# Autodesk Inventor assembly: GP9-100
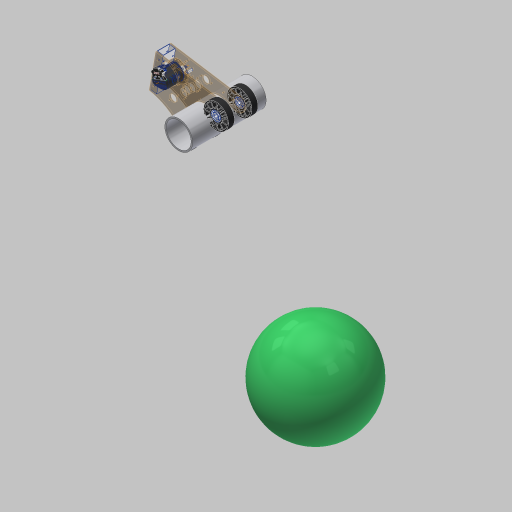
[picture p0: Inventor's stored thumbnail of the model, 512x512]
Saved by Autodesk Inventor 2023.5 (Build 275446000, 446)
## iProperties
Created: 2025-02-27
Part Number: GP9-100
Document SubType Name: Assembly
Designer: dlangdon
Author: dlangdon
## Documents named in this file (11)
- C:\Users\slick\OneDrive\Desktop\2025-ReefScape---CAD\Gripper\GP9\GP9-100.iam
- C:\Users\slick\OneDrive\Desktop\2025-ReefScape---CAD\Gripper\GP9\GP9-001.ipt
- C:\Users\slick\OneDrive\Desktop\2025-ReefScape---CAD\Gripper\GP9\GP9-002.ipt
- C:\Users\slick\OneDrive\Desktop\2025-ReefScape---CAD\Gripper\GP9\GP9-004.ipt
- C:\Users\slick\OneDrive\Desktop\2025-ReefScape---CAD\Gripper\GP9\GP9-003.ipt
- C:\Users\slick\OneDrive\Desktop\2025-ReefScape---CAD\Gripper\GP6\GP6-006.ipt
- C:\Users\slick\OneDrive\Desktop\2025-ReefScape---CAD\COMMON PARTS\MOTORS\Kracken with Cover and Boards.iam
- C:\Users\slick\OneDrive\Desktop\2025-ReefScape---CAD\COMMON PARTS\PULLEYS\gt2\16T Falcon GT216T x 9mm Wide Double Flange Aluminum Pulley (GT2 3mm, Falcon Motor)  (217-6924).iam
- C:\Users\slick\OneDrive\Desktop\2025-ReefScape---CAD\COMMON PARTS\WHEELS\am-3480 4IN 500Hex Bore Compliant Wheel REV2 (1).iam
- C:\Users\slick\OneDrive\Desktop\2025-ReefScape---CAD\Field Items\Game Pieces\GE-25500.ipt
- C:\Users\slick\OneDrive\Desktop\2025-ReefScape---CAD\Field Items\Game Pieces\GE-25501.ipt
## Components (14 placed, 10 different names)
1. GP9-001:1 — Insert:1, Insert:2, Insert:7, Insert:8, Mate:1, Mate:4
2. GP9-002:1 — Insert:3, Insert:4, Mate:2, Mate:3, Mate:5
3. GP9-004:1 — Insert:1, Insert:2, Insert:3, Insert:4
4. GP9-003:1 — Insert:5, Insert:6, Insert:10, Insert:11
5. GP6-006:1 — Insert:6, Insert:7
6. GP6-006:2 — Insert:5, Insert:8
7. Kracken with Cover and Boards:1 [sub-assembly] — Insert:9, Insert:10, Insert:11
8. 16T Falcon GT216T x 9mm Wide Double Flange Aluminum Pulley (GT2 3mm, Falcon Motor)  (217-6924):1 [sub-assembly] — Insert:9
9. am-3480 4IN 500Hex Bore Compliant Wheel REV2 (1):1 [sub-assembly] — Mate:3, Flush:1
10. am-3480 4IN 500Hex Bore Compliant Wheel REV2 (1):2 [sub-assembly] — Mate:2, Flush:1
11. am-3480 4IN 500Hex Bore Compliant Wheel REV2 (1):3 [sub-assembly] — Mate:1, Flush:2
12. am-3480 4IN 500Hex Bore Compliant Wheel REV2 (1):4 [sub-assembly] — Mate:4, Flush:2
13. GE-25500:1 — Mate:5
14. GE-25501:1
## Relationships (18: Insert 11, Mate 5, Flush 2)
- Insert:1: GP9-001:1 ↔ GP9-004:1
- Insert:2: GP9-001:1 ↔ GP9-004:1
- Insert:3: GP9-002:1 ↔ GP9-004:1
- Insert:4: GP9-002:1 ↔ GP9-004:1
- Insert:5: GP9-003:1 ↔ GP6-006:2
- Insert:6: GP9-003:1 ↔ GP6-006:1
- Insert:7: GP9-001:1 ↔ GP6-006:1
- Insert:8: GP9-001:1 ↔ GP6-006:2
- Insert:9: Kracken with Cover and Boards:1 ↔ 16T Falcon GT216T x 9mm Wide Double Flange Aluminum Pulley (GT2 3mm, Falcon Motor)  (217-6924):1
- Insert:10: GP9-003:1 ↔ Kracken with Cover and Boards:1
- Insert:11: GP9-003:1 ↔ Kracken with Cover and Boards:1
- Mate:1: GP9-001:1 ↔ am-3480 4IN 500Hex Bore Compliant Wheel REV2 (1):3
- Mate:2: GP9-002:1 ↔ am-3480 4IN 500Hex Bore Compliant Wheel REV2 (1):2
- Mate:3: GP9-002:1 ↔ am-3480 4IN 500Hex Bore Compliant Wheel REV2 (1):1
- Mate:4: GP9-001:1 ↔ am-3480 4IN 500Hex Bore Compliant Wheel REV2 (1):4
- Flush:1: am-3480 4IN 500Hex Bore Compliant Wheel REV2 (1):1 ↔ am-3480 4IN 500Hex Bore Compliant Wheel REV2 (1):2
- Flush:2: am-3480 4IN 500Hex Bore Compliant Wheel REV2 (1):3 ↔ am-3480 4IN 500Hex Bore Compliant Wheel REV2 (1):4
- Mate:5: GP9-002:1 ↔ GE-25500:1
